# Autodesk Inventor assembly: 202.004.01_Kraftlimitierung
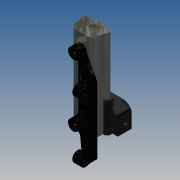
[picture p0: Inventor's stored thumbnail of the model, 180x180]
Saved by Autodesk Inventor 2021 (Build 250183000, 183)
## iProperties
Created: 2021-11-14
Part Number: 202.004.01_Kraftlimitierung
Document SubType Name: Assembly
Designer: Oliver Ungerer
KODE_ZEICHNUNGSNUMMER: TFVEM_121M
BENENNUNG: Kraftlimitierung
BEARBEITER_NAME: Ungerer O.
MATERIAL: PLA gruen
MASSE: 0.070963
PROI_CREATED_BY: Kantioler_adm
PROI_CREATED_ON: 07.03.2008 12:11:19
PROI_LOCATION: Root-Ordner/Pro_stds/Start_Files
EINHEIT: ST
HERSTELLER_PREIS: 0.0
PRUEFER_NAME: Uo
PTC_ORGANIZATION_ID: Durst
PTC_WM_ITERATION: 0
PTC_WM_VERSION: .0
PTC_WM_CREATED_ON: 17.10.21
PTC_WM_MODIFIED_ON: 17.10.21
AEND_INDEX: 0
PTC_MODIFIED: True
PDMREV: 0+
PROI_VERSION: 0+
Author: Oliver Ungerer
## Documents named in this file (5)
- E:\Dokumente\MCI-Mechatronik\Master\Semester_3\Projekt_2_Neu\106_Vereinzelungseinheit\206.004.02_Kraftlimitierung.iam
- E:\Dokumente\MCI-Mechatronik\Master\Semester_3\Projekt_2_Neu\106_Vereinzelungseinheit\106.026.01_Fuehrung_Kraftlimitierung.ipt
- E:\Dokumente\MCI-Mechatronik\Master\Semester_3\Projekt_2_Neu\106_Vereinzelungseinheit\106.031.01_Aufnahme_Aktor.ipt
- E:\Dokumente\MCI-Mechatronik\Master\Semester_3\Projekt_2_Neu\106_Vereinzelungseinheit\106.032.01_Aufnahme_Kraftlimitierung.ipt
- E:\Dokumente\MCI-Mechatronik\Master\Semester_3\Projekt_2_Neu\106_Vereinzelungseinheit\106.028.01_Fuehrungsbolzen_Feder.ipt
## Components (4 placed, 4 different names)
1. 106.030.01_Fuehrung_Kraftlimitierung — Passend:3, Passend:4, Passend:5, Passend:6, Passend:7, Fluchtend:1, Passend:8, Passend:9
2. 106.031.01_Aufnahme_Aktor — Passend:6, Passend:7, Fluchtend:1
3. 106.032.01_Aufnahme_Kraftlimitierung — Passend:3, Passend:8, Passend:9
4. 106.033.01_Fuehrungsbolzen_Feder — Passend:4, Passend:5
## Relationships (8: Mate 7, Flush 1)
- Passend:3 [Mate]: 106.030.01_Fuehrung_Kraftlimitierung ↔ 106.032.01_Aufnahme_Kraftlimitierung
- Passend:4 [Mate]: 106.030.01_Fuehrung_Kraftlimitierung ↔ 106.033.01_Fuehrungsbolzen_Feder
- Passend:5 [Mate]: 106.030.01_Fuehrung_Kraftlimitierung ↔ 106.033.01_Fuehrungsbolzen_Feder
- Passend:6 [Mate]: 106.030.01_Fuehrung_Kraftlimitierung ↔ 106.031.01_Aufnahme_Aktor
- Passend:7 [Mate]: 106.030.01_Fuehrung_Kraftlimitierung ↔ 106.031.01_Aufnahme_Aktor
- Fluchtend:1 [Flush]: 106.030.01_Fuehrung_Kraftlimitierung ↔ 106.031.01_Aufnahme_Aktor
- Passend:8 [Mate]: 106.030.01_Fuehrung_Kraftlimitierung ↔ 106.032.01_Aufnahme_Kraftlimitierung
- Passend:9 [Mate]: 106.030.01_Fuehrung_Kraftlimitierung ↔ 106.032.01_Aufnahme_Kraftlimitierung
